# Autodesk Inventor assembly: UpperBody
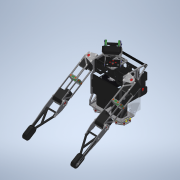
[picture p0: Inventor's stored thumbnail of the model, 180x180]
Saved by Autodesk Inventor 2020.4 (Build 244396000, 396)
## iProperties
Created: 2016-05-03
Part Number: UpperBody
Document SubType Name: Assembly
Designer: hiroaki
Mass: 1684.21 g
Surface Area: 5710.79 cm^2
Volume: 1053.68 cm^3
Density: 1.59841 g/cm^3
Author: hiroaki
## Documents named in this file (9)
- C:\Users\Masato\Documents\Inventor\CIT Brains_Inventor\OpenPlatform_ver3_0 - ve4_1 branch\UpperBody\UpperBody.iam
- C:\Users\Masato\Documents\Inventor\CIT Brains_Inventor\OpenPlatform_ver3_0 - ve4_1 branch\UpperBody\Arm\ForeArm.iam
- C:\Users\Masato\Documents\Inventor\CIT Brains_Inventor\OpenPlatform_ver3_0 - ve4_1 branch\UpperBody\Arm\Shoulder.iam
- C:\Users\Masato\Documents\Inventor\CIT Brains_Inventor\OpenPlatform_ver3_0 - ve4_1 branch\UpperBody\Arm\UpperArm.iam
- C:\Users\Masato\Documents\Inventor\CIT Brains_Inventor\OpenPlatform_ver3_0 - ve4_1 branch\UpperBody\Arm\UpperArm_MIR.iam
- C:\Users\Masato\Documents\Inventor\CIT Brains_Inventor\OpenPlatform_ver3_0 - ve4_1 branch\UpperBody\Head\Head_.iam
- C:\Users\Masato\Documents\Inventor\CIT Brains_Inventor\OpenPlatform_ver3_0 - ve4_1 branch\UpperBody\UpperBody_.iam
- C:\Users\Masato\Documents\Inventor\CIT Brains_Inventor\OpenPlatform_ver3_0 - ve4_1 branch\UpperBody\Cockpit\Cockpit_.iam
- C:\Users\Masato\Documents\Inventor\CIT Brains_Inventor\OpenPlatform_ver3_0 - ve4_1 branch\Ready_Made\Screw\SPNFL-BRN-M3-6.ipt
## Components (11 placed, 8 different names)
1. ForeArm:1 [sub-assembly] — 挿入:102, 挿入:103, 角度:27
2. Shoulder:1 [sub-assembly] — 角度:23, 挿入:100, 挿入:101, 挿入:104
3. Shoulder:2 [sub-assembly] — 角度:23, 挿入:96, 挿入:97, 角度:25, 挿入:105
4. UpperArm_MIR:1 [sub-assembly] — 挿入:96, 挿入:97, 挿入:98, 挿入:99, 角度:25, 角度:26
5. ForeArm:2 [sub-assembly] — 挿入:98, 挿入:99, 角度:26
6. UpperArm:1 [sub-assembly] — 挿入:100, 挿入:101, 挿入:102, 挿入:103, 角度:27
7. Head_:1 [sub-assembly] — 挿入:106
8. UpperBody_:1 [sub-assembly] — 挿入:104, 挿入:105, 挿入:106, フラッシュ:1, フラッシュ:2, フラッシュ:3, 挿入:107, 角度:28, 挿入:108, 挿入:109
9. Cockpit_:1 [sub-assembly] — 挿入:107, 角度:28
10. SPNFL-BRN-M3-6:1 — 挿入:108
11. SPNFL-BRN-M3-6:2 — 挿入:109
## Relationships (22: Insert 14, Angle 5, Flush 3)
- 角度:23 [Angle] (0 deg): Shoulder:1 ↔ Shoulder:2
- 挿入:96 [Insert]: Shoulder:2 ↔ UpperArm_MIR:1
- 挿入:97 [Insert]: Shoulder:2 ↔ UpperArm_MIR:1
- 挿入:98 [Insert]: UpperArm_MIR:1 ↔ ForeArm:2
- 挿入:99 [Insert]: UpperArm_MIR:1 ↔ ForeArm:2
- 挿入:100 [Insert]: Shoulder:1 ↔ UpperArm:1
- 挿入:101 [Insert]: Shoulder:1 ↔ UpperArm:1
- 挿入:102 [Insert]: ForeArm:1 ↔ UpperArm:1
- 挿入:103 [Insert]: ForeArm:1 ↔ UpperArm:1
- 角度:25 [Angle] (0 deg): Shoulder:2 ↔ UpperArm_MIR:1
- 角度:26 [Angle] (0 deg): UpperArm_MIR:1 ↔ ForeArm:2
- 角度:27 [Angle] (0 deg): ForeArm:1 ↔ UpperArm:1
- 挿入:104 [Insert]: Shoulder:1 ↔ UpperBody_:1
- 挿入:105 [Insert]: Shoulder:2 ↔ UpperBody_:1
- 挿入:106 [Insert]: Head_:1 ↔ UpperBody_:1
- フラッシュ:1 [Flush]: UpperBody_:1
- フラッシュ:2 [Flush]: UpperBody_:1
- フラッシュ:3 [Flush]: UpperBody_:1
- 挿入:107 [Insert] (0.25 mm): UpperBody_:1 ↔ Cockpit_:1
- 角度:28 [Angle] (0 deg): UpperBody_:1 ↔ Cockpit_:1
- 挿入:108 [Insert]: UpperBody_:1 ↔ SPNFL-BRN-M3-6:1
- 挿入:109 [Insert]: UpperBody_:1 ↔ SPNFL-BRN-M3-6:2
